# Autodesk Inventor assembly: Additional_Building
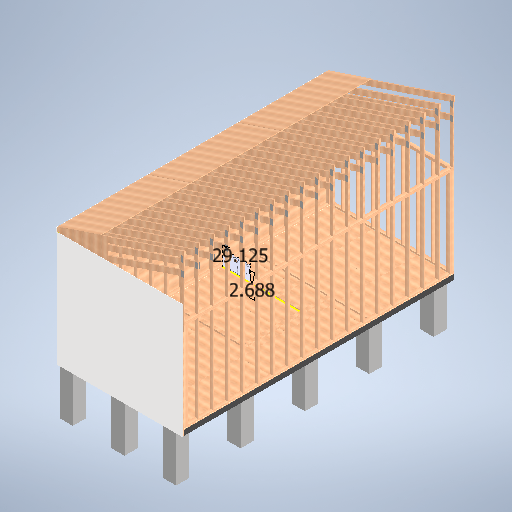
[picture p0: Inventor's stored thumbnail of the model, 512x512]
Saved by Autodesk Inventor 2025.1 (Build 291241020, 241B)
## iProperties
Created: 2024-08-02
Part Number: Additional_Building
Document SubType Name: Assembly
Designer: Tom
Author: Tom
## Documents named in this file (22)
- C:\Users\Tom\Documents\Inventor\Mobility\Additional_Building\Additional_Building.iam
- C:\Users\Tom\Documents\Inventor\Mobility\Additional_Building\Grid_Of_Piers.iam
- C:\Users\Tom\Documents\Inventor\Mobility\Additional_Building\Floor_System.iam
- C:\Users\Tom\Documents\Inventor\Mobility\Additional_Building\Walls.iam
- C:\Users\Tom\Documents\Inventor\Mobility\Additional_Building\Truss.iam
- C:\Users\Tom\Documents\Inventor\Mobility\Additional_Building\OSB_For_Walls_With_Dimensions_48_x_96_Inches.ipt
- C:\Users\Tom\Documents\Inventor\Mobility\Additional_Building\OSB_For_Walls_With_Dimensions_48_x_48_Inches.ipt
- C:\Users\Tom\Documents\Inventor\Mobility\Additional_Building\OSB_For_Roof_With_Dimensions_96_x_48.ipt
- C:\Users\Tom\Documents\Inventor\Mobility\Additional_Building\OSB_For_Walls_With_Dimensions_25.5_x_96_Inches.ipt
- C:\Users\Tom\Documents\Inventor\Mobility\Additional_Building\Block_With_Width_13.75_Inches.ipt
- C:\Users\Tom\Documents\Inventor\Mobility\Additional_Building\Block_With_Width_14.5_Inches.ipt
- C:\Users\Tom\Documents\Inventor\Mobility\Additional_Building\DensGlass_With_Dimensions_36.5_x_48_Inches.ipt
- C:\Users\Tom\Documents\Inventor\Mobility\Additional_Building\DensGlass_With_Dimensions_48_x_96_Inches.ipt
- C:\Users\Tom\Documents\Inventor\Mobility\Additional_Building\DensGlass_With_Dimensions_48_x_84.5_Inches.ipt
- C:\Users\Tom\Documents\Inventor\Mobility\Additional_Building\DensGlass_With_Dimensions_60.75_x_12_Inches.ipt
- C:\Users\Tom\Documents\Inventor\Mobility\Additional_Building\DensGlass_With_Dimensions_36.5_x_25.5_Inches.ipt
- C:\Users\Tom\Documents\Inventor\Mobility\Additional_Building\DensGlass_With_Dimensions_25.5_x_96_Inches.ipt
- C:\Users\Tom\Documents\Inventor\Mobility\Additional_Building\Siding_For_Back_Wall.iam
- C:\Users\Tom\Documents\Inventor\Mobility\Additional_Building\Fascia.ipt
- C:\Users\Tom\Documents\Inventor\Mobility\Additional_Building\OSB_For_Walls_With_Dimensions_36.5_x_96_Inches.ipt
- C:\Users\Tom\Documents\Inventor\Mobility\Additional_Building\OSB_For_Side_And_Back.ipt
- C:\Users\Tom\Documents\Inventor\Mobility\Additional_Building\Siding_For_Side_Wall.iam
## Components (77 placed, 21 different names)
1. Grid_Of_Piers:1 [sub-assembly] — Mate:1, Flush:1, Mate:2
2. Floor_System:1 [sub-assembly] — Mate:1, Flush:1, Mate:2, Mate:3, Flush:2, Flush:3, Flush:15, Flush:16, Flush:29, Flush:30, Flush:31, Flush:33, Mate:51, Flush:41, Mate:53, Flush:42, Mate:55, Flush:44
3. Walls:1 [sub-assembly] — Mate:3, Flush:2, Flush:3, Flush:4, Flush:5, Mate:4, Flush:7, Mate:5, Mate:9, Mate:10, Flush:17, Mate:12, Mate:15, Mate:18, Flush:43
4. OSB_For_Walls_With_Dimensions_48_x_48_Inches:1 — Mate:10, Mate:11, Flush:17, Mate:13, Mate:34
5. OSB_For_Walls_With_Dimensions_48_x_48_Inches:2 — Mate:15, Mate:16, Mate:17, Mate:29, Flush:32
6. Block_With_Width_13.75_Inches:1 — Mate:21, Flush:22, Flush:23
7. Block_With_Width_13.75_Inches:2 — Flush:26, Mate:23, Flush:27, Flush:39
8. DensGlass_With_Dimensions_36.5_x_48_Inches:1 — Mate:24, Flush:28, Flush:29, Mate:26
9. DensGlass_With_Dimensions_36.5_x_48_Inches:2 — Mate:27, Mate:28, Flush:31
10. DensGlass_With_Dimensions_48_x_84.5_Inches:1 — Mate:29, Flush:32, Mate:30, Mate:32, Mate:38, Mate:41, Mate:44
11. DensGlass_With_Dimensions_48_x_96_Inches:3 — Mate:31, Mate:32, Mate:33, Mate:35
12. DensGlass_With_Dimensions_48_x_84.5_Inches:2 — Mate:34, Mate:35, Mate:36, Mate:47
13. DensGlass_With_Dimensions_36.5_x_25.5_Inches:1 — Mate:39, Mate:40, Mate:41, Mate:43
14. DensGlass_With_Dimensions_36.5_x_25.5_Inches:2 — Mate:45, Mate:46, Mate:47
15. Siding_For_Back_Wall:1 [sub-assembly] — Mate:48, Flush:34, Flush:35
16. OSB_For_Walls_With_Dimensions_48_x_96_Inches:6 — Mate:51, Mate:52, Flush:41, Mate:54, Mate:58, Mate:59
17. OSB_For_Walls_With_Dimensions_48_x_96_Inches:7 — Mate:53, Mate:54, Flush:42
18. OSB_For_Walls_With_Dimensions_36.5_x_96_Inches:1 — Mate:55, Flush:43, Flush:44, Flush:45
19. OSB_For_Side_And_Back:1 — Mate:56, Mate:57, Mate:58
20. Siding_For_Side_Wall:1 [sub-assembly] — Mate:59, Mate:60, Flush:45
21. Truss:1 [sub-assembly] — Flush:6, Mate:23, Flush:27, Mate:50, Flush:40, Mate:56
22. Truss:2 [sub-assembly] — Flush:4, Flush:5, Mate:4, Mate:20, Mate:49, Flush:36, Flush:37
23. Truss:3 [sub-assembly] — Flush:6, Flush:7, Mate:5, Flush:26
24. Truss:4 [sub-assembly]
25. Truss:5 [sub-assembly]
26. Truss:6 [sub-assembly]
27. Truss:7 [sub-assembly]
28. Truss:8 [sub-assembly]
29. Truss:9 [sub-assembly]
30. Truss:10 [sub-assembly]
31. Truss:11 [sub-assembly]
32. Truss:12 [sub-assembly]
33. Truss:13 [sub-assembly]
34. Truss:14 [sub-assembly]
35. Truss:15 [sub-assembly]
36. Truss:16 [sub-assembly]
37. Truss:17 [sub-assembly]
38. Truss:18 [sub-assembly] — Mate:22, Flush:25
39. Truss:19 [sub-assembly] — Mate:21, Flush:22, Flush:23, Flush:24
40. OSB_For_Roof_With_Dimensions_96_x_48:1
41. OSB_For_Roof_With_Dimensions_96_x_48:2
42. OSB_For_Roof_With_Dimensions_96_x_48:3 — Mate:49, Flush:36, Flush:37
43. OSB_For_Walls_With_Dimensions_48_x_96_Inches:1 — Mate:9, Flush:15, Flush:16, Mate:11, Mate:16, Flush:18, Mate:24, Flush:28, Mate:25, Mate:37
44. OSB_For_Walls_With_Dimensions_48_x_96_Inches:2
45. OSB_For_Walls_With_Dimensions_48_x_96_Inches:3 — Mate:14, Mate:27
46. OSB_For_Walls_With_Dimensions_48_x_96_Inches:4 — Mate:12, Mate:13, Mate:14, Mate:31
47. OSB_For_Walls_With_Dimensions_48_x_96_Inches:5 — Mate:17
48. OSB_For_Walls_With_Dimensions_25.5_x_96_Inches:1 — Mate:18, Flush:18, Mate:20, Mate:39
49. OSB_For_Walls_With_Dimensions_25.5_x_96_Inches:2 — Mate:42
50. OSB_For_Walls_With_Dimensions_25.5_x_96_Inches:3 — Mate:45
51. Block_With_Width_14.5_Inches:1 — Flush:24, Mate:22, Flush:25
52. Block_With_Width_14.5_Inches:2
53. Block_With_Width_14.5_Inches:3
54. Block_With_Width_14.5_Inches:4
55. Block_With_Width_14.5_Inches:5
56. Block_With_Width_14.5_Inches:6
57. Block_With_Width_14.5_Inches:7
58. Block_With_Width_14.5_Inches:8
59. Block_With_Width_14.5_Inches:9
60. Block_With_Width_14.5_Inches:10
61. Block_With_Width_14.5_Inches:11
62. Block_With_Width_14.5_Inches:12
63. Block_With_Width_14.5_Inches:13
64. Block_With_Width_14.5_Inches:14
65. Block_With_Width_14.5_Inches:15
66. Block_With_Width_14.5_Inches:16
67. DensGlass_With_Dimensions_48_x_96_Inches:1 — Mate:25, Mate:26, Flush:30, Mate:30, Mate:33
68. DensGlass_With_Dimensions_48_x_96_Inches:2 — Mate:28, Mate:36
69. DensGlass_With_Dimensions_60.75_x_12_Inches:1 — Mate:37, Mate:38, Flush:33
70. DensGlass_With_Dimensions_60.75_x_12_Inches:2 — Mate:48, Flush:34, Flush:35, Mate:52
71. DensGlass_With_Dimensions_60.75_x_12_Inches:3 — Mate:40
72. DensGlass_With_Dimensions_60.75_x_12_Inches:4 — Mate:57
73. DensGlass_With_Dimensions_25.5_x_96_Inches:1 — Mate:42, Mate:43, Mate:44
74. DensGlass_With_Dimensions_25.5_x_96_Inches:2 — Mate:46
75. Fascia:1 — Mate:50, Flush:39, Flush:40, Mate:60
76. Fascia:2
77. Fascia:3
## Component patterns: (2 elements, first: Truss:1), (17 elements, first: Truss:3), (3 elements, first: OSB_For_Roof_With_Dimensions_96_x_48:1), (3 elements, first: OSB_For_Walls_With_Dimensions_48_x_96_Inches:1), (2 elements, first: OSB_For_Walls_With_Dimensions_48_x_96_Inches:4), (3 elements, first: OSB_For_Walls_With_Dimensions_25.5_x_96_Inches:1), (16 elements, first: Block_With_Width_14.5_Inches:1), (2 elements, first: DensGlass_With_Dimensions_48_x_96_Inches:1), (4 elements, first: DensGlass_With_Dimensions_60.75_x_12_Inches:1), (2 elements, first: DensGlass_With_Dimensions_25.5_x_96_Inches:1), (3 elements, first: Fascia:1)
## Relationships (90: Mate 56, Flush 34)
- Mate:1: Grid_Of_Piers:1 ↔ Floor_System:1
- Flush:1: Grid_Of_Piers:1 ↔ Floor_System:1
- Mate:2: Grid_Of_Piers:1 ↔ Floor_System:1
- Mate:3: Floor_System:1 ↔ Walls:1
- Flush:2: Floor_System:1 ↔ Walls:1
- Flush:3: Floor_System:1 ↔ Walls:1
- Flush:4: Walls:1 ↔ Truss:2
- Flush:5: Walls:1 ↔ Truss:2
- Mate:4: Walls:1 ↔ Truss:2
- Flush:6 (387.35 mm): Truss:1 ↔ Truss:3
- Flush:7: Walls:1 ↔ Truss:3
- Mate:5: Walls:1 ↔ Truss:3
- Mate:9: Walls:1 ↔ OSB_For_Walls_With_Dimensions_48_x_96_Inches:1
- Flush:15: Floor_System:1 ↔ OSB_For_Walls_With_Dimensions_48_x_96_Inches:1
- Flush:16: Floor_System:1 ↔ OSB_For_Walls_With_Dimensions_48_x_96_Inches:1
- Mate:10: Walls:1 ↔ OSB_For_Walls_With_Dimensions_48_x_48_Inches:1
- Mate:11: OSB_For_Walls_With_Dimensions_48_x_48_Inches:1 ↔ OSB_For_Walls_With_Dimensions_48_x_96_Inches:1
- Flush:17: Walls:1 ↔ OSB_For_Walls_With_Dimensions_48_x_48_Inches:1
- Mate:12: Walls:1 ↔ OSB_For_Walls_With_Dimensions_48_x_96_Inches:4
- Mate:13: OSB_For_Walls_With_Dimensions_48_x_48_Inches:1 ↔ OSB_For_Walls_With_Dimensions_48_x_96_Inches:4
- Mate:14: OSB_For_Walls_With_Dimensions_48_x_96_Inches:3 ↔ OSB_For_Walls_With_Dimensions_48_x_96_Inches:4
- Mate:15: Walls:1 ↔ OSB_For_Walls_With_Dimensions_48_x_48_Inches:2
- Mate:16: OSB_For_Walls_With_Dimensions_48_x_48_Inches:2 ↔ OSB_For_Walls_With_Dimensions_48_x_96_Inches:1
- Mate:17: OSB_For_Walls_With_Dimensions_48_x_48_Inches:2 ↔ OSB_For_Walls_With_Dimensions_48_x_96_Inches:5
- Mate:18: Walls:1 ↔ OSB_For_Walls_With_Dimensions_25.5_x_96_Inches:1
- Flush:18: OSB_For_Walls_With_Dimensions_48_x_96_Inches:1 ↔ OSB_For_Walls_With_Dimensions_25.5_x_96_Inches:1
- Mate:20: Truss:2 ↔ OSB_For_Walls_With_Dimensions_25.5_x_96_Inches:1
- Mate:21: Block_With_Width_13.75_Inches:1 ↔ Truss:19
- Flush:22: Block_With_Width_13.75_Inches:1 ↔ Truss:19
- Flush:23: Block_With_Width_13.75_Inches:1 ↔ Truss:19
- Flush:24: Truss:19 ↔ Block_With_Width_14.5_Inches:1
- Mate:22: Truss:18 ↔ Block_With_Width_14.5_Inches:1
- Flush:25: Truss:18 ↔ Block_With_Width_14.5_Inches:1
- Flush:26: Block_With_Width_13.75_Inches:2 ↔ Truss:3
- Mate:23: Block_With_Width_13.75_Inches:2 ↔ Truss:1
- Flush:27: Block_With_Width_13.75_Inches:2 ↔ Truss:1
- Mate:24: DensGlass_With_Dimensions_36.5_x_48_Inches:1 ↔ OSB_For_Walls_With_Dimensions_48_x_96_Inches:1
- Flush:28 (292.1 mm): DensGlass_With_Dimensions_36.5_x_48_Inches:1 ↔ OSB_For_Walls_With_Dimensions_48_x_96_Inches:1
- Flush:29: Floor_System:1 ↔ DensGlass_With_Dimensions_36.5_x_48_Inches:1
- Mate:25: OSB_For_Walls_With_Dimensions_48_x_96_Inches:1 ↔ DensGlass_With_Dimensions_48_x_96_Inches:1
- Mate:26: DensGlass_With_Dimensions_36.5_x_48_Inches:1 ↔ DensGlass_With_Dimensions_48_x_96_Inches:1
- Flush:30: Floor_System:1 ↔ DensGlass_With_Dimensions_48_x_96_Inches:1
- Mate:27: DensGlass_With_Dimensions_36.5_x_48_Inches:2 ↔ OSB_For_Walls_With_Dimensions_48_x_96_Inches:3
- Mate:28: DensGlass_With_Dimensions_36.5_x_48_Inches:2 ↔ DensGlass_With_Dimensions_48_x_96_Inches:2
- Flush:31: Floor_System:1 ↔ DensGlass_With_Dimensions_36.5_x_48_Inches:2
- Mate:29: OSB_For_Walls_With_Dimensions_48_x_48_Inches:2 ↔ DensGlass_With_Dimensions_48_x_84.5_Inches:1
- Flush:32 (292.1 mm): OSB_For_Walls_With_Dimensions_48_x_48_Inches:2 ↔ DensGlass_With_Dimensions_48_x_84.5_Inches:1
- Mate:30: DensGlass_With_Dimensions_48_x_84.5_Inches:1 ↔ DensGlass_With_Dimensions_48_x_96_Inches:1
- Mate:31: DensGlass_With_Dimensions_48_x_96_Inches:3 ↔ OSB_For_Walls_With_Dimensions_48_x_96_Inches:4
- Mate:32: DensGlass_With_Dimensions_48_x_84.5_Inches:1 ↔ DensGlass_With_Dimensions_48_x_96_Inches:3
- Mate:33: DensGlass_With_Dimensions_48_x_96_Inches:3 ↔ DensGlass_With_Dimensions_48_x_96_Inches:1
- Mate:34: OSB_For_Walls_With_Dimensions_48_x_48_Inches:1 ↔ DensGlass_With_Dimensions_48_x_84.5_Inches:2
- Mate:35: DensGlass_With_Dimensions_48_x_96_Inches:3 ↔ DensGlass_With_Dimensions_48_x_84.5_Inches:2
- Mate:36: DensGlass_With_Dimensions_48_x_84.5_Inches:2 ↔ DensGlass_With_Dimensions_48_x_96_Inches:2
- Mate:37: OSB_For_Walls_With_Dimensions_48_x_96_Inches:1 ↔ DensGlass_With_Dimensions_60.75_x_12_Inches:1
- Mate:38: DensGlass_With_Dimensions_48_x_84.5_Inches:1 ↔ DensGlass_With_Dimensions_60.75_x_12_Inches:1
- Flush:33: Floor_System:1 ↔ DensGlass_With_Dimensions_60.75_x_12_Inches:1
- Mate:39: DensGlass_With_Dimensions_36.5_x_25.5_Inches:1 ↔ OSB_For_Walls_With_Dimensions_25.5_x_96_Inches:1
- Mate:40: DensGlass_With_Dimensions_36.5_x_25.5_Inches:1 ↔ DensGlass_With_Dimensions_60.75_x_12_Inches:3
- Mate:41: DensGlass_With_Dimensions_48_x_84.5_Inches:1 ↔ DensGlass_With_Dimensions_36.5_x_25.5_Inches:1
- Mate:42: OSB_For_Walls_With_Dimensions_25.5_x_96_Inches:2 ↔ DensGlass_With_Dimensions_25.5_x_96_Inches:1
- Mate:43: DensGlass_With_Dimensions_36.5_x_25.5_Inches:1 ↔ DensGlass_With_Dimensions_25.5_x_96_Inches:1
- Mate:44: DensGlass_With_Dimensions_48_x_84.5_Inches:1 ↔ DensGlass_With_Dimensions_25.5_x_96_Inches:1
- Mate:45: DensGlass_With_Dimensions_36.5_x_25.5_Inches:2 ↔ OSB_For_Walls_With_Dimensions_25.5_x_96_Inches:3
- Mate:46: DensGlass_With_Dimensions_36.5_x_25.5_Inches:2 ↔ DensGlass_With_Dimensions_25.5_x_96_Inches:2
- Mate:47: DensGlass_With_Dimensions_48_x_84.5_Inches:2 ↔ DensGlass_With_Dimensions_36.5_x_25.5_Inches:2
- Mate:48: Siding_For_Back_Wall:1 ↔ DensGlass_With_Dimensions_60.75_x_12_Inches:2
- Flush:34: Siding_For_Back_Wall:1 ↔ DensGlass_With_Dimensions_60.75_x_12_Inches:2
- Flush:35: Siding_For_Back_Wall:1 ↔ DensGlass_With_Dimensions_60.75_x_12_Inches:2
- Mate:49: Truss:2 ↔ OSB_For_Roof_With_Dimensions_96_x_48:3
- Flush:36: Truss:2 ↔ OSB_For_Roof_With_Dimensions_96_x_48:3
- Flush:37: Truss:2 ↔ OSB_For_Roof_With_Dimensions_96_x_48:3
- Mate:50: Truss:1 ↔ Fascia:1
- Flush:39 (-12.319 mm): Block_With_Width_13.75_Inches:2 ↔ Fascia:1
- Flush:40 (-30.3276 mm): Truss:1 ↔ Fascia:1
- Mate:51: Floor_System:1 ↔ OSB_For_Walls_With_Dimensions_48_x_96_Inches:6
- Mate:52: OSB_For_Walls_With_Dimensions_48_x_96_Inches:6 ↔ DensGlass_With_Dimensions_60.75_x_12_Inches:2
- Flush:41: Floor_System:1 ↔ OSB_For_Walls_With_Dimensions_48_x_96_Inches:6
- Mate:53: Floor_System:1 ↔ OSB_For_Walls_With_Dimensions_48_x_96_Inches:7
- Mate:54: OSB_For_Walls_With_Dimensions_48_x_96_Inches:6 ↔ OSB_For_Walls_With_Dimensions_48_x_96_Inches:7
- Flush:42: Floor_System:1 ↔ OSB_For_Walls_With_Dimensions_48_x_96_Inches:7
- Mate:55: Floor_System:1 ↔ OSB_For_Walls_With_Dimensions_36.5_x_96_Inches:1
- Flush:43: Walls:1 ↔ OSB_For_Walls_With_Dimensions_36.5_x_96_Inches:1
- Flush:44: Floor_System:1 ↔ OSB_For_Walls_With_Dimensions_36.5_x_96_Inches:1
- Mate:56: OSB_For_Side_And_Back:1 ↔ Truss:1
- Mate:57: OSB_For_Side_And_Back:1 ↔ DensGlass_With_Dimensions_60.75_x_12_Inches:4
- Mate:58: OSB_For_Walls_With_Dimensions_48_x_96_Inches:6 ↔ OSB_For_Side_And_Back:1
- Mate:59: OSB_For_Walls_With_Dimensions_48_x_96_Inches:6 ↔ Siding_For_Side_Wall:1
- Mate:60: Siding_For_Side_Wall:1 ↔ Fascia:1
- Flush:45 (-6.35 mm): OSB_For_Walls_With_Dimensions_36.5_x_96_Inches:1 ↔ Siding_For_Side_Wall:1
